# Autodesk Inventor assembly: SR-094-D
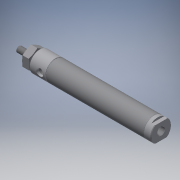
[picture p0: Inventor's stored thumbnail of the model, 180x180]
Saved by Autodesk Inventor 2016 SP1 (Build 200210100, 210)
## iProperties
Category: PARTsolutions
Company: BIMBA
Created: 2017-03-15
Part Number: SR-094-D
Catalog Web Link: www.cadenas.de
Description: Original Line Standard Air Cylinders-
Vendor: BIMBA
Document SubType Name: Assembly
Designer: 589013
Manufacturer: BIMBA
PSOL_IDENT_0: {$CADENAS_DATA\23d-libs\bimba\bimba\bimba_imperial\bimba_full_line\original_line_cylinders\standard_
PSOL_IDENT_1: air_cylinders\standard_air_cylinder_asmtab.prj},316 {VTYP=3D},{STYP=ASSTAB},{NB=SR-094-D},{LINA=SR-0
PSOL_IDENT_2: 94-D},{NN=Original Line Standard Air Cylinders},{DATE=09.11.2016 07:55:11},{GEOMDATE=11.07.2016 10:3
PSOL_IDENT_3: 7:18},{VERSION=},{LINEID=10},{LINESUBID=-1},{WBVAR=STROKE,ACTING,MNT,DER,NR,BM,CO,OO,VO,M,EE,EEL,K,Q
PSOL_IDENT_4: ,Y,G,T,B,H,SER,SR,NT,W,HL,STPT1,STPT2,STPT3,STPT4,MB,PB,PRC,TB,MN}  {NB=SR-094-D},{LINA=SR-094-D},{K
PSOL_IDENT_5: T=DUMMY},{PN=SR-094-D},{PNC=SR-094-D},{PNA=(NO ACCESSORIES)},{DASH=-},{BORE1=1.06250000},{BORE=1 1/1
PSOL_IDENT_6: 6\" (09)},{BOREPN=09},{STROKE=4.000},{STROKEALG=[0.011:50/0.001]},{STROKE1=4.000},{ACTING=D},{ACTING
PSOL_IDENT_7: ALG= '' , 'Single Acting (SA)' , 'R' , 'Reverse Single Acting (SA)' , 'D' , 'Double Acting (SA)' },{
PSOL_IDENT_8: ACTINGPN=D},{MNT=},{MNTALG= '' , 'Front Nose Mounting (SA)' , 'P' , 'Rear Pivot Mounting (SA)' , 'X'
PSOL_IDENT_9: , 'Universal Pivot Mounting or Double End Mounting (SA)' , 'BF' , 'Front Block Mounting (SA)' , 'BR'
PSOL_IDENT_10: , 'Rear Block Mounting for Vertical Positioning (SA)' , 'BFT' , 'Front Block Trunnion Mounting (SA)'
PSOL_IDENT_11: , 'BRT' , 'Rear Block Trunnion Mounting (SA)' },{TYPE=SR-},{MNTPN=},{DER=},{DERALG= '' , 'N/A' },{N
PSOL_IDENT_12: R=},{NRALG= '' , 'N/A' },{NRPN=},{BM=},{BMALG= '' , 'N/A' },{BMPN=},{CO=},{COALG= '' , 'N/A' },{OO=}
PSOL_IDENT_13: ,{OOALG= '', 'N/A' },{OOPN=},{VO=Z},{VOALG= 'Z' , 'N/A' },{VOPN=},{OOVOPN=},{M=},{MALG= '', 'Without
PSOL_IDENT_14: Magnet', 'M', 'With Magnet' },{EE=},{EEL=0.000},{EEMAX=46.0000},{EEALG= '', 'Without Extra Extensio
PSOL_IDENT_15: n', 'EE', 'With Extra Extension' },{EELALG=0},{EEPN=},{EEPN1=0.000},{K=},{KALG= '' , 'N/A' },{KPN=},
PSOL_IDENT_16: {Q=},{QALG= '' , 'Standard Port' , 'Q' , 'Side Port' },{QPN=},{Y=},{YALG= '' , 'N/A' },{YPN=},{YCON=
PSOL_IDENT_17: },{F=},{FALG= '', 'Non-Coated (Standard)', 'F', 'Molycoated' },{FPN=},{G=},{GPN=},{GPN99=},{T=},{TAL
PSOL_IDENT_18: G= '' , 'Standard -20° to 200°F (-29° to 95°C)' , 'N' , 'Low Temperature' , 'V' , 'High Temperature'
PSOL_IDENT_19: },{NPN=},{VPN=},{B=},{BALG= '', 'W/out Bumpers' , 'B' , 'W/ Bumpers' },{BPN=},{H=},{HALG= '', 'N/A'
PSOL_IDENT_20: },{HPN=},{SER=},{SERALG= '' , 'Without Spring Extend/Return' , 'JS' , 'With Spring Return' , 'JR' ,
PSOL_IDENT_21: 'With Spring Extend' },{SR=SR},{SRALG= 'C' , 'Standard Blackened Carbon Steel' , 'SR' , 'Stainless
PSOL_IDENT_22: Steel [SR]' },{SRPN=SR},{SRCON=1},{NT=},{NTPN=},{W=},{WALG= '' , 'Without Wiper' , 'W' , 'With Wiper'
PSOL_IDENT_23: },{WPN=},{E=},{EALG= '' , 'Standard Seals/Lube' , 'E' , 'Non-Lube Seals/Lube' },{EPN=},{HL=},{HLALG=
PSOL_IDENT_24: '' , 'Without Low Pressure Hydraulic' , 'HL' , 'With Low Pressure Hydraulic' },{ST=},{STALG= '' , '
PSOL_IDENT_25: N/A' },{STPT1=},{STPT1ALG= '' , 'N/A' },{STPT2=},{STPT2ALG= '' , 'N/A' },{STPT3=},{STPT3ALG= '' , 'N
PSOL_IDENT_26: /A' },{STPT4=},{STPT4ALG= '' , 'N/A' },{STPN=},{MB=},{MBALG= '' , 'Without Mounting Bracket' , 'F,D-
PSOL_IDENT_27: 129' , 'D-129 (front)' },{MBPN=},{MBPNALL=D-129},{MBPNALLREAR=},{PB=},{PBALG= '' , 'N/A' },{PBPN=},{
PSOL_IDENT_28: PBPNALL=},{PRC=},{PRCALG= '' , 'W/out Pivot Rod Clevis' , 'F,D-166-1' , 'D-166-1 (front)' },{PRCPN=}
PSOL_IDENT_29: ,{PRCPNALL=D-166-1},{TB=},{TBALG= '' , 'N/A' },{TBPN=},{TBPNALL=},{MN=},{MNALG= '' , 'N/A' },{MNPN=}
PSOL_IDENT_30: ,{MNCONF=},{MNCONR=},{TLEN=5.3125},{FRAC=22.1200},{RGCON=},{RGDACCON=R},{RHCON=},{RHCON1=},{RHCONON=
PSOL_IDENT_31: 1},{RHACCON=},{FNUTCON=1},{RNUTCON=0},{FNUTPN=D-9},{RNUTPN=},{FNUTTRANS=0.0000},{RNUTTRANS=0.0000},{
PSOL_IDENT_32: VHOLECON=0},{A1=1.6250},{A1N=1.0000},{A1P=1.6250},{A1B=1.8750},{A4=0.2525},{A4N=0.3750},{A4P=0.2525}
PSOL_IDENT_33: ,{A5=0.0300},{A1H=0.625},{A1NH=0.6250},{A1PH=1.5000},{A1BH=1.1250},{A1SH=1.1250},{A2H=0.2500},{A2NH=
PSOL_IDENT_34: 0.2500},{LENGTH=3.1200},{LENGTH1=3.1200},{LENGTH2=3.3800},{MUL=4.0000},{MUL11=4.0000},{MUL22=10.24},
PSOL_IDENT_35: {MUL33=6.2400},{MUL2=4.0000},{MUL211=4.0000},{MUL222=2.5600},{MUL233=1.5600},{SSS=8.0000},{RGLEN=1.4
PSOL_IDENT_36: 025},{RHLEN=0.4050},{SSS1=5.0000},{A13=1.2190},{DIF=0.0000},{G5=0.7180},{ON=0},{SSADD=0.1250},{BADD=
PSOL_IDENT_37: 0.0000},{MADD=0.0000},{NVADD=0.0000},{TRACKL=5.0225},{TRACKCON=D-78527},{TRIMCON=0},{TRIMCON1=0},{PI
PSOL_IDENT_38: NCON=},{FSPACE=0.8069},{SPACE=0.1214},{TEXT=0.2125},{S1=1.2500},{D1=1.1410},{D1N=1.1130},{D1B=1.1130
PSOL_IDENT_39: },{D1P=1.1410},{FA=0.940},{RA=0.9400},{PPATH=standard_air_cylinder_asmtpl.prj},{MATALGHTML=<b>Standa
PSOL_IDENT_40: rd Original Line:</b><dl><dt>Rod:</dt><dd>- Stainless Steel</dd><dd>&nbsp;&nbsp;(5/16 9/16 Bores)</d
PSOL_IDENT_41: d><dd>- High Strength Carbon Steel</dd><dd>&nbsp;&nbsp;(3/4 3 Bore)</dd><dd>- Stainless Steel</dd><d
PSOL_IDENT_42: d>&nbsp;&nbsp;(X style DXP/DX/DXDE)</dd><dt>Bearings:</dt><dd>- Sintered Bronze</dd><dt>Body:</dt><d
PSOL_IDENT_43: d>- 304 Stainless Steel</dd><dt>End Caps:</dt><dd>- Aluminum</dd><dt>Seals:</dt><dd>- Buna N</dd></d
PSOL_IDENT_44: l>},{ASSCFGPRA=09D},{MBPNA=},{MNPNA=},{PRCPNA=},{ASSOPTACC=STPT4},{A=7.25},{HADD=0.0000},{WFL=0.125}
PSOL_IDENT_45: ,{QADD=0.000},{QADD1=0.250},{TEST=4.0000},{MNTB=},{STDNUTF=1},{STDNUTR=0},{STRK2D=0},{X2D=2},{STROKE
PSOL_IDENT_46: SW=4.000},{EESW=0.000},{FCD=0},{BCD=0},{RCD=0},{CUSTADD=3.000},{FT=5/16-24 UNF-2A},{FT1=5/16-24 UNF-
PSOL_IDENT_47: 2A},{FT2=5/8-18 UNF-2A},{PORT=1/8 NPT},{FT11=5/8-18 UNF-2A},{FT12=5/8-18 UNF-2A}
NN: Original Line Standard Air Cylinders
NT: Standard Male Thread
NB: SR-094-D
NBSYN: $PNC.
LINA: SR-094-D
PN: SR-094-D
PNA: (NO ACCESSORIES)
BORE: 1 1/16" [09]
STROKE: 4.000
ACTING: Double [D]
MNT: Standard Front Nose
DER: N/A
NR: N/A
BM: N/A
CO: N/A
OO: N/A
VO: N/A
M: Without Magnet Piston
EE: Standard Rod Extension
EEL: 0.000
K: N/A
Q: Standard Axial Port
Y: N/A
G: Standard Grease Lube
T: Standard -20° to 200°F (-29° to 95°C)
B: Without Bumpers
H: N/A
SER: Without Failsafe Spring Extend/Return
SR: Stainless Steel [SR]
W: Without Wiper
HL: Standard 250 PSI Air
STPT1: N/A
STPT2: N/A
STPT3: N/A
STPT4: N/A
MB: Without Mounting Bracket
PB: N/A
PRC: Without Piston Rod Clevis
TB: N/A
MN: N/A
A: 7.25
SUPPLIER: BIMBA
ARTICLENO: SR-094-D
BOMINFO: SR-094-D
CREATOR: CADENAS GmbH
Title: SR-094-D
Author: Cadenas PARTsolutions
## Documents named in this file (7)
- E:\Pneumatics Shtuff\SR-094-D\SR-094-D.iam
- E:\Pneumatics Shtuff\SR-094-D\SR-094-DSR0000_0_dummy.ipt
- E:\Pneumatics Shtuff\SR-094-D\09R000-0_rod_guide.ipt
- E:\Pneumatics Shtuff\SR-094-D\09R-5_31250SR.ipt
- E:\Pneumatics Shtuff\SR-094-D\090000_rear_head.ipt
- E:\Pneumatics Shtuff\SR-094-D\D-9.ipt
- E:\Pneumatics Shtuff\SR-094-D\SR-094-D0_rod.ipt
## Components (6 placed, 6 different names)
1. SR-094-DSR0000_0_dummy:1 — dummy_XY@1 <-> rod_guide_XY@2, dummy_Z@1 <-> rod_guide_Z@2, dummy_YZ@1 <-> rod_guide_YZ@2
2. 09R000-0_rod_guide:1 — dummy_XY@1 <-> rod_guide_XY@2, dummy_Z@1 <-> rod_guide_Z@2, dummy_YZ@1 <-> rod_guide_YZ@2, to_tube_XY@2 <-> tube_front_XY@3, to_tube_Z@2 <-> tube_front_Z@3, to_tube_YZ@2 <-> tube_front_YZ@3, to_nut_XY@2 <-> NUT_XY@5, to_nut_Z@2 <-> NUT_Z@5, to_nut_YZ@2 <-> NUT_YZ@5, to_rod_XY@2 <-> rod_cp_XY@6, to_rod_Z@2 <-> rod_cp_Z@6
3. 09R-5_31250SR:1 — to_tube_XY@2 <-> tube_front_XY@3, to_tube_Z@2 <-> tube_front_Z@3, to_tube_YZ@2 <-> tube_front_YZ@3, tube_rear_XY@3 <-> to_tube_XY@4, tube_rear_Z@3 <-> to_tube_Z@4, tube_rear_YZ@3 <-> to_tube_YZ@4
4. 090000_rear_head:1 — tube_rear_XY@3 <-> to_tube_XY@4, tube_rear_Z@3 <-> to_tube_Z@4, tube_rear_YZ@3 <-> to_tube_YZ@4
5. D-9:1 — to_nut_XY@2 <-> NUT_XY@5, to_nut_Z@2 <-> NUT_Z@5, to_nut_YZ@2 <-> NUT_YZ@5
6. SR-094-D0_rod:1 — to_rod_XY@2 <-> rod_cp_XY@6, to_rod_Z@2 <-> rod_cp_Z@6
## Relationships (14: Flush 5, Mate 5, Angle 4)
- dummy_XY@1 <-> rod_guide_XY@2 [Flush]: SR-094-DSR0000_0_dummy:1 ↔ 09R000-0_rod_guide:1
- dummy_Z@1 <-> rod_guide_Z@2 [Mate]: SR-094-DSR0000_0_dummy:1 ↔ 09R000-0_rod_guide:1
- dummy_YZ@1 <-> rod_guide_YZ@2 [Angle] (0 deg): SR-094-DSR0000_0_dummy:1 ↔ 09R000-0_rod_guide:1
- to_tube_XY@2 <-> tube_front_XY@3 [Flush]: 09R000-0_rod_guide:1 ↔ 09R-5_31250SR:1
- to_tube_Z@2 <-> tube_front_Z@3 [Mate]: 09R000-0_rod_guide:1 ↔ 09R-5_31250SR:1
- to_tube_YZ@2 <-> tube_front_YZ@3 [Angle] (0 deg): 09R000-0_rod_guide:1 ↔ 09R-5_31250SR:1
- tube_rear_XY@3 <-> to_tube_XY@4 [Flush]: 09R-5_31250SR:1 ↔ 090000_rear_head:1
- tube_rear_Z@3 <-> to_tube_Z@4 [Mate]: 09R-5_31250SR:1 ↔ 090000_rear_head:1
- tube_rear_YZ@3 <-> to_tube_YZ@4 [Angle] (0 deg): 09R-5_31250SR:1 ↔ 090000_rear_head:1
- to_nut_XY@2 <-> NUT_XY@5 [Flush]: 09R000-0_rod_guide:1 ↔ D-9:1
- to_nut_Z@2 <-> NUT_Z@5 [Mate]: 09R000-0_rod_guide:1 ↔ D-9:1
- to_nut_YZ@2 <-> NUT_YZ@5 [Angle] (0 deg): 09R000-0_rod_guide:1 ↔ D-9:1
- to_rod_XY@2 <-> rod_cp_XY@6 [Flush]: 09R000-0_rod_guide:1 ↔ SR-094-D0_rod:1
- to_rod_Z@2 <-> rod_cp_Z@6 [Mate]: 09R000-0_rod_guide:1 ↔ SR-094-D0_rod:1
